# Autodesk Inventor assembly: Assembly1
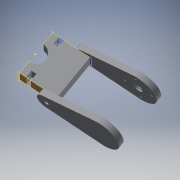
[picture p0: Inventor's stored thumbnail of the model, 180x180]
Saved by Autodesk Inventor 2018 (Build 220112000, 112)
## iProperties
Created: 2017-06-05
Part Number: Assembly1
Document SubType Name: Assembly
Designer: Zadeka
Author: Zadeka
## Documents named in this file (4)
- C:\Users\Zadeka\Desktop\Assembly1.iam
- C:\Users\Zadeka\Desktop\BIKE.ipt
- C:\Users\Zadeka\Desktop\motormount.ipt
- C:\Users\Zadeka\Desktop\Part2.ipt
## Components (3 placed, 3 different names)
1. BIKE:1 — Rotational:1, Rotational:2
2. motormount:1 — Rotational:2, Mate:1
3. Part2:1 — Rotational:1, Mate:1
## Relationships (3: RevoluteJoint 2, Mate 1)
- Rotational:1 [RevoluteJoint]: BIKE:1 ↔ Part2:1
- Rotational:2 [RevoluteJoint]: BIKE:1 ↔ motormount:1
- Mate:1: motormount:1 ↔ Part2:1
